# Autodesk Inventor assembly: BasisRoboter
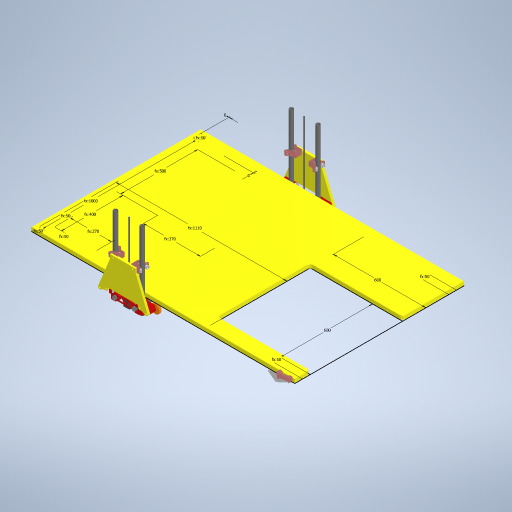
[picture p0: Inventor's stored thumbnail of the model, 512x512]
Saved by Autodesk Inventor 2024 (Build 280153000, 153)
## iProperties
Created: 2023-11-24
Part Number: BasisRoboter
Document SubType Name: Assembly
Designer: danie
Author: danie
## Documents named in this file (7)
- C:\GitHubDesktop\3d-model\basis_roboter\BasisRoboter.iam
- C:\GitHubDesktop\3d-model\basis_roboter\Grundplatte.ipt
- C:\GitHubDesktop\3d-model\basis_roboter\low_rider_v2\custom_files\XY_Assemblie.iam
- C:\GitHubDesktop\3d-model\Y_Pipe.ipt
- C:\GitHubDesktop\3d-model\basis_roboter\low_rider_v2\custom_files\Slead_Assemblie.iam
- C:\GitHubDesktop\3d-model\Imported Components\Belt_Stop\Belt_Stop.ipt
- C:\GitHubDesktop\3d-model\basis_roboter\Saugknopf.ipt
## Components (8 placed, 6 different names)
1. Grundplatte:1 — Slider:1, Mate:1, Mate:2, Flush:1, Flush:2
2. Y_Pipe:1 — Rigid:2
3. Y_Pipe:2 — Cylindrical:1, Rigid:1, Cylindrical:2
4. Slead_Assemblie:1 [sub-assembly] — Cylindrical:2
5. Belt_Stop:1 — Slider:1
6. XY_Assemblie:1 [sub-assembly] — Mate:1, Flush:1, Rigid:1, Rigid:2
7. XY_Assemblie:2 [sub-assembly] — Mate:2, Flush:2, Cylindrical:1
8. Saugknopf:1
## Relationships (9: Mate 2, Flush 2, CylindricalJoint 2, WeldJoint 2, TranslationJoint 1)
- Slider:1 [TranslationJoint]: Grundplatte:1 ↔ Belt_Stop:1
- Mate:1 (45 mm): Grundplatte:1 ↔ XY_Assemblie:1
- Mate:2 (45 mm): Grundplatte:1 ↔ XY_Assemblie:2
- Flush:1 (-8 mm): Grundplatte:1 ↔ XY_Assemblie:1
- Flush:2 (-8 mm): Grundplatte:1 ↔ XY_Assemblie:2
- Cylindrical:1: Y_Pipe:2 ↔ XY_Assemblie:2
- Rigid:1 [WeldJoint]: Y_Pipe:2 ↔ XY_Assemblie:1
- Rigid:2 [WeldJoint]: Y_Pipe:1 ↔ XY_Assemblie:1
- Cylindrical:2: Y_Pipe:2 ↔ Slead_Assemblie:1
